# Autodesk Inventor assembly: StartAssembly
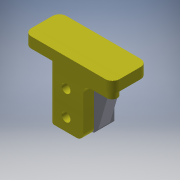
[picture p0: Inventor's stored thumbnail of the model, 180x180]
Saved by Autodesk Inventor 2018 (Build 220112000, 112)
## iProperties
Created: 2020-05-13
Part Number: StartAssembly
Document SubType Name: Assembly
Designer: Ivan
Author: Ivan
## Documents named in this file (3)
- C:\Users\Ivan\Documents\GitHub\AR_CODEX\3DModels\StartAssembly.iam
- C:\Users\Ivan\Documents\GitHub\AR_CODEX\3DModels\EndSwitch.ipt
- C:\Users\Ivan\Documents\GitHub\AR_CODEX\3DModels\StartSupport.ipt
## Components (2 placed, 2 different names)
1. EndSwitch:1 — Mate:1, Mate:2, Mate:3
2. StartSupport:1 — Mate:1, Mate:2, Mate:3
## Relationships (3: Mate 3)
- Mate:1: EndSwitch:1 ↔ StartSupport:1
- Mate:2: EndSwitch:1 ↔ StartSupport:1
- Mate:3: EndSwitch:1 ↔ StartSupport:1
